# Autodesk Inventor assembly: Anglerfish
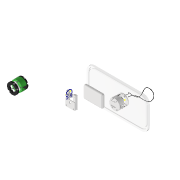
[picture p0: Inventor's stored thumbnail of the model, 180x180]
Saved by Autodesk Inventor 2022 (Build 260153000, 153)
## iProperties
Created: 2022-04-02
Part Number: Anglerfish
Document SubType Name: Assembly
Designer: Prakash Lab
Author: Prakash Lab
## Documents named in this file (16)
- C:\Users\diederichbenedict\Dropbox\Dokumente\Promotion\PROJECTS\Matchboxscope\INVENTOR\RELEASE\Anglerfish\Workspace\Anglerfish.iam
- C:\Users\diederichbenedict\Dropbox\Dokumente\Promotion\PROJECTS\Matchboxscope\INVENTOR\RELEASE\Anglerfish\Workspace\00_ESP3-CAM.iam
- C:\Users\diederichbenedict\Dropbox\Dokumente\Promotion\PROJECTS\Matchboxscope\INVENTOR\RELEASE\Anglerfish\Workspace\00_Powerbank.ipt
- C:\Users\diederichbenedict\Dropbox\Dokumente\Promotion\PROJECTS\Matchboxscope\INVENTOR\RELEASE\InjectionMolded\Matchboxscope_M12_Lensadapter_v0.ipt
- C:\Users\diederichbenedict\Dropbox\Dokumente\Promotion\PROJECTS\Matchboxscope\INVENTOR\RELEASE\InjectionMolded\00_CCTV_M12_VCM_large.ipt
- C:\Users\diederichbenedict\Dropbox\Dokumente\Promotion\PROJECTS\Matchboxscope\INVENTOR\RELEASE\Anglerfish\Workspace\Anglerfish_flipped_LidMoun.ipt
- C:\Users\diederichbenedict\Dropbox\Dokumente\Promotion\PROJECTS\Matchboxscope\INVENTOR\RELEASE\Anglerfish\Workspace\Anglerfish_flipped_Electronicsmount.ipt
- C:\Users\diederichbenedict\Dropbox\Dokumente\Promotion\PROJECTS\Matchboxscope\INVENTOR\RELEASE\Anglerfish\Workspace\00_Magnet_8x3mm.ipt
- C:\Users\diederichbenedict\Dropbox\Dokumente\Promotion\PROJECTS\Matchboxscope\INVENTOR\RELEASE\Anglerfish\Workspace\DIN 912 - M3 x 0.5 x 12 x 10.75.ipt
- C:\Users\diederichbenedict\Dropbox\Dokumente\Promotion\PROJECTS\Matchboxscope\INVENTOR\RELEASE\Anglerfish\Workspace\00_Toslink.ipt
- C:\Users\diederichbenedict\Dropbox\Dokumente\Promotion\PROJECTS\Matchboxscope\INVENTOR\RELEASE\Anglerfish\Workspace\00_lunchbox_body.ipt
- C:\Users\diederichbenedict\Dropbox\Dokumente\Promotion\PROJECTS\Matchboxscope\INVENTOR\RELEASE\Anglerfish\Workspace\00_Lunchbox_cover.ipt
- C:\Users\diederichbenedict\Dropbox\Dokumente\Promotion\PROJECTS\Matchboxscope\INVENTOR\RELEASE\Anglerfish\Workspace\Anglerfish_coverslipclamp_top.ipt
- C:\Users\diederichbenedict\Dropbox\Dokumente\Promotion\PROJECTS\Matchboxscope\INVENTOR\RELEASE\Anglerfish\Workspace\Anglerfish_coverslipclamp_levelarm.ipt
- C:\Users\diederichbenedict\Dropbox\Dokumente\Promotion\PROJECTS\Matchboxscope\INVENTOR\RELEASE\Anglerfish\Workspace\Anglerfish_coverslipclamp_lampclamp.ipt
- C:\Users\diederichbenedict\Dropbox\Dokumente\Promotion\PROJECTS\Matchboxscope\INVENTOR\RELEASE\InjectionMolded\Assembly_Matchboxscope_injectionmolded_Anglerfish.iam
## Components (27 placed, 15 different names)
1. 00_Powerbank:1
2. 00_ESP3-CAM:1 [sub-assembly] — Winkel:11
3. 00_CCTV_M12_VCM_large:1 — Passend:30, Einfügen:11
4. Matchboxscope_M12_Lensadapter_v0:1 — Einfügen:11
5. Anglerfish_flipped_Electronicsmount:1 — Winkel:11, Passend:30
6. 00_Magnet_8x3mm:2 — Einfügen:21
7. 00_Magnet_8x3mm:3
8. 00_Magnet_8x3mm:4 — Einfügen:20
9. 00_Magnet_8x3mm:5
10. 00_Magnet_8x3mm:6
11. DIN 912 - replaced by DIN EN ISO 4762 M3 x 12:1
12. DIN 912 - replaced by DIN EN ISO 4762 M3 x 12:2
13. DIN 912 - replaced by DIN EN ISO 4762 M3 x 12:4
14. DIN 912 - replaced by DIN EN ISO 4762 M3 x 12:5
15. DIN 912 - replaced by DIN EN ISO 4762 M3 x 12:6
16. DIN 912 - replaced by DIN EN ISO 4762 M3 x 12:7
17. 00_Toslink:1
18. 00_lunchbox_body:1 — Fluchtend:4, Winkel:14, Fluchtend:33, Fluchtend:34, Passend:31
19. 00_Lunchbox_cover:1 — Fluchtend:33, Fluchtend:34, Passend:31, Fluchtend:35
20. Anglerfish_flipped_LidMoun:1 — Fluchtend:35, Einfügen:19, Einfügen:20, Einfügen:21
21. 00_Magnet_8x3mm:7 — Einfügen:19
22. Matchboxscope_M12_Lensadapter_v0:2
23. 00_Powerbank:2
24. Anglerfish_coverslipclamp_top:1 — Fluchtend:36, Fluchtend:37, Fluchtend:38, Fluchtend:39
25. Anglerfish_coverslipclamp_levelarm:1 — Fluchtend:36, Fluchtend:37
26. Anglerfish_coverslipclamp_lampclamp:1 — Fluchtend:38, Fluchtend:39
27. Assembly_Matchboxscope_injectionmolded_Anglerfish:1 [sub-assembly]
## Relationships (16: Flush 8, Insert 4, Angle 2, Mate 2)
- Winkel:11 [Angle] (180 deg): 00_ESP3-CAM:1 ↔ Anglerfish_flipped_Electronicsmount:1
- Passend:30 [Mate]: 00_CCTV_M12_VCM_large:1 ↔ Anglerfish_flipped_Electronicsmount:1
- Einfügen:11 [Insert]: 00_CCTV_M12_VCM_large:1 ↔ Matchboxscope_M12_Lensadapter_v0:1
- Fluchtend:4 [Flush]: 00_lunchbox_body:1
- Winkel:14 [Angle] (180 deg): 00_lunchbox_body:1
- Fluchtend:33 [Flush]: 00_lunchbox_body:1 ↔ 00_Lunchbox_cover:1
- Fluchtend:34 [Flush]: 00_lunchbox_body:1 ↔ 00_Lunchbox_cover:1
- Passend:31 [Mate]: 00_lunchbox_body:1 ↔ 00_Lunchbox_cover:1
- Fluchtend:35 [Flush] (-5 mm): 00_Lunchbox_cover:1 ↔ Anglerfish_flipped_LidMoun:1
- Einfügen:19 [Insert]: Anglerfish_flipped_LidMoun:1 ↔ 00_Magnet_8x3mm:7
- Einfügen:20 [Insert]: 00_Magnet_8x3mm:4 ↔ Anglerfish_flipped_LidMoun:1
- Einfügen:21 [Insert]: 00_Magnet_8x3mm:2 ↔ Anglerfish_flipped_LidMoun:1
- Fluchtend:36 [Flush]: Anglerfish_coverslipclamp_top:1 ↔ Anglerfish_coverslipclamp_levelarm:1
- Fluchtend:37 [Flush]: Anglerfish_coverslipclamp_top:1 ↔ Anglerfish_coverslipclamp_levelarm:1
- Fluchtend:38 [Flush]: Anglerfish_coverslipclamp_top:1 ↔ Anglerfish_coverslipclamp_lampclamp:1
- Fluchtend:39 [Flush]: Anglerfish_coverslipclamp_top:1 ↔ Anglerfish_coverslipclamp_lampclamp:1
